# Autodesk Inventor assembly: 19
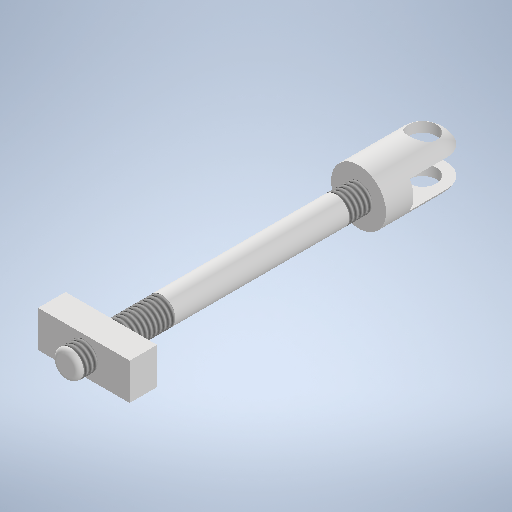
[picture p0: Inventor's stored thumbnail of the model, 512x512]
Saved by Autodesk Inventor 2025.1 (Build 291241000, 241)
## iProperties
Created: 2024-09-13
Part Number: 19
Document SubType Name: Assembly
Designer: ffogue
Author: ffogue
## Documents named in this file (4)
- C:\Users\ffogue\Documents\Inventor\Single cylinder Steam Engine\19.iam
- C:\Users\ffogue\Documents\Inventor\Single cylinder Steam Engine\19.1.ipt
- C:\Users\ffogue\Documents\Inventor\Single cylinder Steam Engine\19.2.ipt
- C:\Users\ffogue\Documents\Inventor\Single cylinder Steam Engine\19.ipt
## Components (3 placed, 3 different names)
1. 19.1:1 — Mate:1, Rotational:1, Angle:1
2. 19.2:1 — Mate:1, Mate:2, Rotational:1, Insert:1
3. 19:1 — Mate:2, Insert:1, Angle:1
## Relationships (5: Mate 2, RevoluteJoint 1, Insert 1, Angle 1)
- Mate:1: 19.1:1 ↔ 19.2:1
- Mate:2: 19.2:1 ↔ 19:1
- Rotational:1 [RevoluteJoint] (-3 mm): 19.1:1 ↔ 19.2:1
- Insert:1 (-5 mm): 19.2:1 ↔ 19:1
- Angle:1 (90 deg): 19.1:1 ↔ 19:1
